# Autodesk Inventor assembly: Montagem
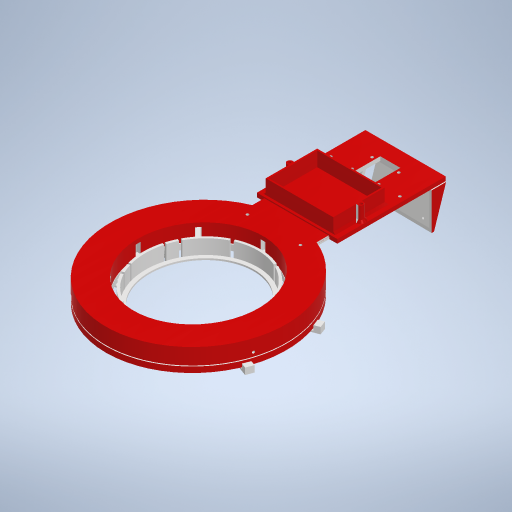
[picture p0: Inventor's stored thumbnail of the model, 512x512]
Saved by Autodesk Inventor 2024.3 (Build 283343000, 343)
## iProperties
Created: 2024-12-01
Part Number: Montagem
Document SubType Name: Assembly
Designer: lostv
Author: lostv
## Documents named in this file (8)
- C:\Users\lostv\OneDrive\Área de Trabalho\modelagens_ic\Montagem_ic.iam
- C:\Users\lostv\OneDrive\Área de Trabalho\modelagens_ic\tampa_anel.ipt
- C:\Users\lostv\OneDrive\Área de Trabalho\modelagens_ic\peca_principal.ipt
- C:\Users\lostv\OneDrive\Área de Trabalho\modelagens_ic\anel.ipt
- C:\Users\lostv\Downloads\16x2-lcd.snapshot.2\LCD.ipt
- C:\Users\lostv\OneDrive\Área de Trabalho\modelagens_ic\tampa_princpal.ipt
- C:\Users\lostv\OneDrive\Área de Trabalho\modelagens_ic\suporte_peca2.ipt
- C:\Users\lostv\OneDrive\Área de Trabalho\modelagens_ic\calibracao(0,5cm).ipt
## Components (7 placed, 7 different names)
1. tampa_anel:2
2. peca_principal:1
3. anel:1
4. LCD:1
5. tampa_princpal:1
6. suporte_peca2:1
7. calibracao(0,5cm):1
## Named parameters: Finish1_Area = 999.153
note: some values were not read from the file. Shown as the stored number, unit unknown: "Finish1_Area".
